# Autodesk Inventor assembly: ShovelAssembly
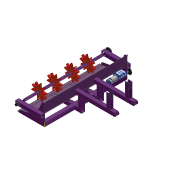
[picture p0: Inventor's stored thumbnail of the model, 180x180]
Saved by Autodesk Inventor 2012 (Build 160160000, 160)
## iProperties
Created: 2013-01-29
Part Number: ShovelAssembly
Document SubType Name: Assembly
Designer: JesseK
Mass: 2585.26 g
Surface Area: 10324.9 cm^2
Volume: 911.712 cm^3
Density: 2.83561 g/cm^3
Author: JesseK
## Documents named in this file (15)
- Z:\UserData\Documents\Inventor\team1885frc\Robot2013\FloorPickup\ShovelAssembly.iam
- Z:\UserData\Documents\Inventor\team1885frc\Robot2013\FloorPickup\Shovel_Arm.ipt
- Z:\UserData\Documents\Inventor\team1885frc\Robot2013\FloorPickup\PivotLeverBar.ipt
- Z:\UserData\Documents\Inventor\team1885frc\Robot2013\FloorPickup\Shovel_VerticalArm.ipt
- Z:\UserData\Documents\Inventor\team1885frc\Robot2013\FloorPickup\Shovel_BottomFrame.ipt
- Z:\UserData\Documents\Inventor\team1885frc\Robot2013\FloorPickup\Shovel_CrossFrame.ipt
- Z:\UserData\Documents\Inventor\team1885frc\Robot2013\FloorPickup\Shovel_Scoop.ipt
- Z:\UserData\Documents\Inventor\team1885frc\VEXPro\VersaPlanetary Gearbox\217-2625 with AM-9015.20121205\217-2625 with AM-9015.20121205.iam
- Z:\UserData\Documents\Inventor\team1885frc\Robot2013\FloorPickup\Shovel_SideWall.ipt
- Z:\UserData\Documents\Inventor\team1885frc\Robot2013\FloorPickup\Shovel_RollerMount.ipt
- Z:\UserData\Documents\Inventor\team1885frc\Robot2013\FloorPickup\IntakeRoller.ipt
- Z:\UserData\Documents\Inventor\team1885frc\Hardware\Bearings\Bearing_0.375ID_0.875OD_flanged.ipt
- Z:\UserData\Documents\Inventor\team1885frc\Robot2013\FloorPickup\Shovel_RollerDriveAxle.ipt
- Z:\UserData\Documents\Inventor\team1885frc\VEXPro\#25 Sprokets\22T-Hub-hex.217-2640.20121204.ipt
- Z:\UserData\Documents\Inventor\team1885frc\Robot2013\FloorPickup\Shovel_RollerAxle.ipt
## Components (26 placed, 14 different names)
1. Shovel_Arm:1 — Mate:1, Flush:1, Mate:2, Flush:3, Mate:4, Flush:4, Mate:8, Mate:9
2. Shovel_Arm:2 — Mate:1, Flush:1, Mate:2, Flush:2, Mate:3, Mate:6, Flush:5, Mate:11
3. PivotLeverBar:1 — Flush:2, Mate:3, Mate:5, Mate:6
4. PivotLeverBar:2 — Flush:3, Mate:4, Mate:5
5. Shovel_VerticalArm:1 — Flush:4, Mate:7, Mate:8, Mate:9, Flush:6, Flush:7, Mate:10, Mate:13
6. Shovel_VerticalArm:2 — Flush:5, Mate:7, Flush:8, Flush:9, Mate:11, Mate:12
7. Shovel_BottomFrame:1 — Flush:6, Flush:7, Mate:10, Flush:11, Mate:14, Mate:15
8. Shovel_BottomFrame:2 — Flush:8, Flush:9, Mate:12, Flush:10
9. Shovel_CrossFrame:1 — Flush:10, Flush:11, Mate:13, Flush:12, Flush:13, Flush:14, Mate:17, Mate:18, Mate:19, Mate:20
10. Shovel_Scoop:1 — Flush:12, Flush:13, Mate:14, Mate:15, Flush:15, Flush:16, Mate:16, Flush:17
11. 217-2625 with AM-9015.20121205:1 [sub-assembly] — Flush:14, Mate:17, Mate:18, Mate:34
12. Shovel_SideWall:1 — Flush:15, Flush:16, Mate:20, Mate:21
13. Shovel_SideWall:2 — Mate:16, Flush:17, Mate:19, Flush:18, Flush:19, Mate:26
14. Shovel_RollerMount:1 — Flush:18, Mate:22, Mate:23, Mate:25, Flush:19, Mate:26, Mate:27, Mate:28
15. Shovel_RollerMount:2 — Mate:21, Mate:22, Mate:23, Mate:29, Mate:30, Mate:47
16. IntakeRoller:1 — Mate:25, Mate:39, Mate:40, Mate:49
17. Bearing_0.375ID_0.875OD_flanged:1 — Mate:27, Mate:28, Mate:31, Mate:32, Mate:35
18. Bearing_0.375ID_0.875OD_flanged:2 — Mate:29, Mate:30, Mate:37, Mate:38
19. Shovel_RollerDriveAxle:1 — Mate:31, Mate:32, Mate:33, Tangent:1, Tangent:2, Mate:36
20. 22T-Hub-hex.217-2640.20121204:1 — Mate:33, Flush:20, Mate:35
21. 22T-Hub-hex.217-2640.20121204:2 — Mate:34, Flush:20
22. Shovel_RollerAxle:1 — Tangent:1, Tangent:2, Mate:36, Mate:39, Mate:40, Mate:41, Mate:42, Mate:43, Mate:44, Mate:45, Mate:46
23. Shovel_RollerDriveAxle:2 — Mate:37, Mate:38
24. IntakeRoller:2 — Mate:41, Mate:44, Mate:49
25. IntakeRoller:3 — Mate:42, Mate:45, Mate:48
26. IntakeRoller:4 — Mate:43, Mate:46, Mate:47, Mate:48
## Relationships (70: Mate 48, Flush 20, Tangent 2)
- Mate:1: Shovel_Arm:1 ↔ Shovel_Arm:2
- Flush:1: Shovel_Arm:1 ↔ Shovel_Arm:2
- Mate:2 (114.3 mm): Shovel_Arm:1 ↔ Shovel_Arm:2
- Flush:2: Shovel_Arm:2 ↔ PivotLeverBar:1
- Flush:3: Shovel_Arm:1 ↔ PivotLeverBar:2
- Mate:3: Shovel_Arm:2 ↔ PivotLeverBar:1
- Mate:4: Shovel_Arm:1 ↔ PivotLeverBar:2
- Mate:5: PivotLeverBar:1 ↔ PivotLeverBar:2
- Mate:6 (31.75 mm): Shovel_Arm:2 ↔ PivotLeverBar:1
- Flush:4: Shovel_Arm:1 ↔ Shovel_VerticalArm:1
- Flush:5: Shovel_Arm:2 ↔ Shovel_VerticalArm:2
- Mate:7: Shovel_VerticalArm:1 ↔ Shovel_VerticalArm:2
- Mate:8: Shovel_Arm:1 ↔ Shovel_VerticalArm:1
- Mate:9 (25.4 mm): Shovel_Arm:1 ↔ Shovel_VerticalArm:1
- Flush:6: Shovel_VerticalArm:1 ↔ Shovel_BottomFrame:1
- Flush:7: Shovel_VerticalArm:1 ↔ Shovel_BottomFrame:1
- Mate:10: Shovel_VerticalArm:1 ↔ Shovel_BottomFrame:1
- Flush:8: Shovel_VerticalArm:2 ↔ Shovel_BottomFrame:2
- Flush:9: Shovel_VerticalArm:2 ↔ Shovel_BottomFrame:2
- Mate:11: Shovel_Arm:2 ↔ Shovel_VerticalArm:2
- Mate:12: Shovel_VerticalArm:2 ↔ Shovel_BottomFrame:2
- Flush:10 (-222.25 mm): Shovel_BottomFrame:2 ↔ Shovel_CrossFrame:1
- Flush:11: Shovel_BottomFrame:1 ↔ Shovel_CrossFrame:1
- Mate:13 (25.4 mm): Shovel_VerticalArm:1 ↔ Shovel_CrossFrame:1
- Flush:12: Shovel_CrossFrame:1 ↔ Shovel_Scoop:1
- Flush:13: Shovel_CrossFrame:1 ↔ Shovel_Scoop:1
- Mate:14: Shovel_BottomFrame:1 ↔ Shovel_Scoop:1
- Mate:15: Shovel_BottomFrame:1 ↔ Shovel_Scoop:1
- Flush:14: Shovel_CrossFrame:1 ↔ 217-2625 with AM-9015.20121205:1
- Flush:15: Shovel_Scoop:1 ↔ Shovel_SideWall:1
- Flush:16: Shovel_Scoop:1 ↔ Shovel_SideWall:1
- Mate:16: Shovel_Scoop:1 ↔ Shovel_SideWall:2
- Flush:17: Shovel_Scoop:1 ↔ Shovel_SideWall:2
- Mate:17: Shovel_CrossFrame:1 ↔ 217-2625 with AM-9015.20121205:1
- Mate:18: Shovel_CrossFrame:1 ↔ 217-2625 with AM-9015.20121205:1
- Mate:19: Shovel_CrossFrame:1 ↔ Shovel_SideWall:2
- Mate:20: Shovel_CrossFrame:1 ↔ Shovel_SideWall:1
- Flush:18: Shovel_SideWall:2 ↔ Shovel_RollerMount:1
- Mate:21: Shovel_SideWall:1 ↔ Shovel_RollerMount:2
- Mate:22: Shovel_RollerMount:1 ↔ Shovel_RollerMount:2
- Mate:23: Shovel_RollerMount:1 ↔ Shovel_RollerMount:2
- Mate:25 (114.3 mm): Shovel_RollerMount:1 ↔ IntakeRoller:1
- Flush:19 (12.7 mm): Shovel_SideWall:2 ↔ Shovel_RollerMount:1
- Mate:26 (-63.5 mm): Shovel_SideWall:2 ↔ Shovel_RollerMount:1
- Mate:27: Shovel_RollerMount:1 ↔ Bearing_0.375ID_0.875OD_flanged:1
- Mate:28: Shovel_RollerMount:1 ↔ Bearing_0.375ID_0.875OD_flanged:1
- Mate:29: Shovel_RollerMount:2 ↔ Bearing_0.375ID_0.875OD_flanged:2
- Mate:30: Shovel_RollerMount:2 ↔ Bearing_0.375ID_0.875OD_flanged:2
- Mate:31: Bearing_0.375ID_0.875OD_flanged:1 ↔ Shovel_RollerDriveAxle:1
- Mate:32: Bearing_0.375ID_0.875OD_flanged:1 ↔ Shovel_RollerDriveAxle:1
- Mate:33: Shovel_RollerDriveAxle:1 ↔ 22T-Hub-hex.217-2640.20121204:1
- Mate:34: 217-2625 with AM-9015.20121205:1 ↔ 22T-Hub-hex.217-2640.20121204:2
- Flush:20: 22T-Hub-hex.217-2640.20121204:1 ↔ 22T-Hub-hex.217-2640.20121204:2
- Mate:35: Bearing_0.375ID_0.875OD_flanged:1 ↔ 22T-Hub-hex.217-2640.20121204:1
- Tangent:1: Shovel_RollerDriveAxle:1 ↔ Shovel_RollerAxle:1
- Tangent:2: Shovel_RollerDriveAxle:1 ↔ Shovel_RollerAxle:1
- Mate:36: Shovel_RollerDriveAxle:1 ↔ Shovel_RollerAxle:1
- Mate:37: Bearing_0.375ID_0.875OD_flanged:2 ↔ Shovel_RollerDriveAxle:2
- Mate:38: Bearing_0.375ID_0.875OD_flanged:2 ↔ Shovel_RollerDriveAxle:2
- Mate:39: IntakeRoller:1 ↔ Shovel_RollerAxle:1
- Mate:40: IntakeRoller:1 ↔ Shovel_RollerAxle:1
- Mate:41: Shovel_RollerAxle:1 ↔ IntakeRoller:2
- Mate:42: Shovel_RollerAxle:1 ↔ IntakeRoller:3
- Mate:43: Shovel_RollerAxle:1 ↔ IntakeRoller:4
- Mate:44: Shovel_RollerAxle:1 ↔ IntakeRoller:2
- Mate:45: Shovel_RollerAxle:1 ↔ IntakeRoller:3
- Mate:46: Shovel_RollerAxle:1 ↔ IntakeRoller:4
- Mate:47 (127 mm): Shovel_RollerMount:2 ↔ IntakeRoller:4
- Mate:48 (101.6 mm): IntakeRoller:3 ↔ IntakeRoller:4
- Mate:49 (101.6 mm): IntakeRoller:1 ↔ IntakeRoller:2
